# Autodesk Inventor assembly: mirror_assembly_70mm
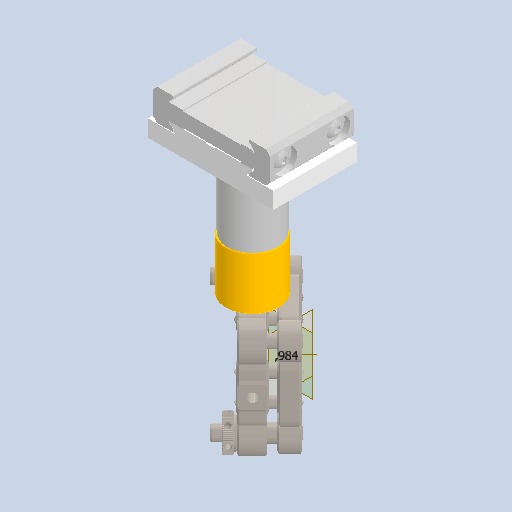
[picture p0: Inventor's stored thumbnail of the model, 512x512]
Saved by Autodesk Inventor 2026.1 (Build 301233000, 233)
## iProperties
Created: 2019-05-24
Part Number: mirror_assembly_70mm
Document SubType Name: Assembly
Designer: Julian
Author: Julian
## Documents named in this file (6)
- C:\Users\user\Desktop\setup for publishing\mirror_assembly_70mm.iam
- C:\Users\user\Desktop\setup for publishing\rail_mount.iam
- C:\Users\user\Desktop\setup for publishing\M-PS-1E_1in_70mm_post.ipt
- C:\Users\user\Desktop\setup for publishing\SS100-F2H_suprema_1in_mirror_mount.ipt
- C:\Users\user\Desktop\setup for publishing\1in_2mm_Quadline.ipt
- C:\Users\user\Desktop\setup for publishing\SM1S1M-1mm_brass_spacer.ipt
## Components (5 placed, 5 different names)
1. rail_mount:1 [sub-assembly] — Mate:5, Mate:6, Angle:1
2. M-PS-1E_1in_70mm_post:1 — Mate:3, Mate:4, Mate:5, Mate:6
3. SS100-F2H_suprema_1in_mirror_mount:1 — Mate:3, Mate:4, Mate:8, Mate:9, Mate:10
4. 1in_2mm_Quadline:1 — Mate:8, Angle:1, Mate:11
5. SM1S1M-1mm_brass_spacer:1 — Mate:9, Mate:10, Mate:11
## Relationships (9: Mate 8, Angle 1)
- Mate:3: M-PS-1E_1in_70mm_post:1 ↔ SS100-F2H_suprema_1in_mirror_mount:1
- Mate:4: M-PS-1E_1in_70mm_post:1 ↔ SS100-F2H_suprema_1in_mirror_mount:1
- Mate:5: rail_mount:1 ↔ M-PS-1E_1in_70mm_post:1
- Mate:6: rail_mount:1 ↔ M-PS-1E_1in_70mm_post:1
- Mate:8: SS100-F2H_suprema_1in_mirror_mount:1 ↔ 1in_2mm_Quadline:1
- Angle:1 (0 deg): rail_mount:1 ↔ 1in_2mm_Quadline:1
- Mate:9: SS100-F2H_suprema_1in_mirror_mount:1 ↔ SM1S1M-1mm_brass_spacer:1
- Mate:10: SS100-F2H_suprema_1in_mirror_mount:1 ↔ SM1S1M-1mm_brass_spacer:1
- Mate:11: 1in_2mm_Quadline:1 ↔ SM1S1M-1mm_brass_spacer:1
